# Autodesk Inventor assembly: Rebuild Shooter Assembly
(part 2 of 2)
- Insert:168: Bearing Mount v1:1 ↔ 91831A411:4
- Insert:169: Bearing Mount v1:1 ↔ 91831A411:5
- Insert:170: Bearing Mount v1:1 ↔ 91831A411:6
- Insert:171: Runner Rails v2:1 ↔ 91735A831:1
- Insert:172: Runner Rails v2:1 ↔ 91735A831:2
- Insert:173: Runner Rails v2:1 ↔ 91735A831:3
- Insert:174: Runner Rails v2:1 ↔ 91735A831:4
- Insert:175: Runner Rails v2:1 ↔ 91735A831:6
- Insert:176: Runner Rails v2:1 ↔ 91735A831:5
- Mate:119: Shooter Top Shield:1 ↔ Shooter Magnetic Sensor Mount Bracket:1
- Angle:74 (5 deg): Shooter Magnetic Sensor Mount Bracket:1 ↔ Bearing Mount Top:1
- Mate:120: Shooter Magnetic Sensor Mount Bracket:1 ↔ Bearing Mount Top:1
- Mate:121 (12.7 mm): Shooter Magnetic Sensor Mount Bracket:1 ↔ Bearing Mount Top:1
- Insert:177: Shooter Magnetic Sensor Mount Bracket:1 ↔ Shooter Magnetic Sensor V2:1
- Insert:178: Shooter Magnetic Sensor Mount Bracket:1 ↔ 7:1
- Insert:179: 7:1 ↔ 7:2
- [Insert]: Shooter Magnetic Sensor Mount Bracket:1 ↔ Standard #4 Washer:15
- [Insert]: Shooter Magnetic Sensor Mount Bracket:1 ↔ Standard #4 Washer:16
- Insert:182: Standard #10 Washer:6 ↔ 91831A411:7
- Insert:183: Standard #10 Washer:7 ↔ 91831A411:8
- Insert:184: Standard #10 Washer:8 ↔ 91831A411:9
- Insert:185: Standard #10 Washer:9 ↔ 91831A411:10
- Insert:186: Standard #10 Washer:10 ↔ 91831A411:11
- Insert:187: Standard #10 Washer:11 ↔ 91831A411:12
- Insert:188: Pneumatic Hub:2 ↔ Standard #10 Washer:6
- Insert:189: Pneumatic Hub:2 ↔ Standard #10 Washer:7
- Insert:190: Pneumatic Hub:2 ↔ Standard #10 Washer:8
- Insert:191: Pneumatic Hub:2 ↔ Standard #10 Washer:9
- Insert:192: Pneumatic Hub:2 ↔ Standard #10 Washer:10
- Insert:193: Pneumatic Hub:2 ↔ Standard #10 Washer:11
- Mate:122 (12.7 mm): Bearing Mount Top:1 ↔ Pneumatic Hub:2
- Flush:73: Shooter Top Shield:1 ↔ Bearing Mount Top:1
- Mate:123: Shooter Top Shield:1 ↔ Bearing Mount Top:1
- Flush:74: Shooter Top Shield:1 ↔ Bearing Mount Top:1
- Flush:75: Shooter Top Shield:1 ↔ Bearing Mount Top:1
- Mate:124: Shooter Wheel Shields Connector Bar:1 ↔ Wheel Shield 2:1
- Mate:125: Shooter Wheel Shields Connector Bar:1 ↔ Wheel Shield 1:1
- Flush:76: Shooter Wheel Shields Connector Bar:1 ↔ Wheel Shield 2:1
- Mate:126: Rebuild Shooter Main Base:1 ↔ 0.25x20 Washer:95
- Mate:127: Rebuild L-Channel Strength:1 ↔ 0.25x20 Washer:95
- Insert:194: 0.25x20 Washer:95 ↔ 90630A110:34
- Insert:195: 92620A540:10 ↔ 0.25x20 Washer:63
- Insert:196: DBK_0820Spacer_am-2243 (modified 3):1 ↔ Rebuild Shooter Main Base:1
- [Insert]: Wheel Shield 2:1 ↔ Standard #4 Washer:19
- [Insert]: Wheel Shield 1:1 ↔ Standard #4 Washer:18
- Mate:128: Shooter Wheel Shields Connector Bar:1 ↔ Shooter Side Support Bar - L:1
- Insert:199: Wheel Shield 1:1 ↔ 0.125 Pop Rivet:1
- Insert:200: Wheel Shield 1:1 ↔ 0.125 Pop Rivet:2
- Insert:201: Wheel Shield 2:1 ↔ 0.125 Pop Rivet:3
- Insert:202: Wheel Shield 2:1 ↔ 0.125 Pop Rivet:4
- [Insert]: Wheel Shield 1:1 ↔ Standard #4 Washer:17
- Insert:204: 0.125 Pop Rivet:5 ↔ Hopper Bracing P1:1
- [Insert]: Standard #4 Washer:40 ↔ Hopper Bracing P1:1
- [Insert]: Standard #4 Washer:41 ↔ Hopper Bracing P1:1
- Insert:207: Rebuild Shooter Main Base:1 ↔ 0.25x20 Washer:96
- Insert:208: Rebuild L-Channel Strength:1 ↔ 90630A110:35
- Insert:209: 0.25x20 Washer:96 ↔ 92620A540:11
- Mate:130: Runner Rails v2:1 ↔ Hopper Bracing P2:1
- Mate:132: Runner Rails v2:1 ↔ Hopper Bracing P3:1
- Flush:78 (-6.35 mm): Runner Rails v2:1 ↔ Hopper Bracing P3:1
- Mate:133: Runner Rails v2:1 ↔ Hopper Bracing P2:1
- Flush:79: Hopper Left Side Leg:1 ↔ Hopper Bracing P2:1
- Mate:134: Hopper Left Side Leg:1 ↔ Hopper Bracing P2:1
- Mate:135: Runner Rails v2:1 ↔ Hopper Left Side Leg:1
- Mate:137: Hopper Left Side Leg:1 ↔ Hopper Bracing P3:1
- Mate:138: Hopper Bracing Right Leg P13:1 ↔ Hopper Right Side Leg:1
- Mate:153: Bearing Mount Top:1 ↔ Hopper Right Side Leg:1
- Mate:140: Hopper Left Side:1 ↔ Hopper Left Side Leg:1
- Flush:81: Hopper Bottom:1 ↔ Hopper Left Side:1
- Mate:141: Hopper Bottom:1 ↔ Hopper Back Wedge Side:1
- Mate:142: Hopper Left Side:1 ↔ Hopper Back Wedge Side:1
- Flush:82: Hopper Bottom:1 ↔ Hopper Back Wedge Side:1
- Mate:143: Hopper Bottom:1 ↔ Hopper Left Side:1
- Mate:144: Hopper Bracing Top Left P4:1 ↔ Hopper Top:1
- Flush:83: Hopper Left Side:1 ↔ Hopper Top:1
- Flush:84: Hopper Left Side:1 ↔ Hopper Top:1
- Mate:145: Hopper Bracing Top Left P4:1 ↔ Hopper Left Side:1
- Mate:146: Hopper Bracing Top Left P4:1 ↔ Hopper Left Side:1
- Insert:210: 0.125 Pop Rivet:6 ↔ Hopper Left Side:1
- Insert:211: 0.125 Pop Rivet:7 ↔ Hopper Left Side:1
- Insert:212: 0.125 Pop Rivet:8 ↔ Hopper Left Side:1
- Insert:213: 0.125 Pop Rivet:9 ↔ Hopper Left Side:1
- Insert:214: 0.125 Pop Rivet:10 ↔ Hopper Left Side:1
- Mate:147: Hopper Front:1 ↔ Hopper Bottom:1
- Mate:156: Hopper Front:1 ↔ Hopper Left Side:1
- Mate:148: Hopper Front:1 ↔ Hopper Bracing Front Top P8:1
- Mate:167 (0.7937 mm): Hopper Right:1 ↔ Hopper Top:1
- Mate:150: Hopper Front:1 ↔ Hopper Right:1
- Flush:87: Hopper Front:1 ↔ Hopper Right:1
- Mate:151 (0.7937 mm): Hopper Right:1 ↔ Hopper Right Side Leg:1
- Insert:215: 0.125 Pop Rivet:11 ↔ Hopper Top:1
- Insert:216: 0.125 Pop Rivet:12 ↔ Hopper Top:1
- Mate:152 (114.3 mm): Runner Rails v2:1 ↔ Hopper Left Side:1
- Flush:151: Shooter Back Support Bar:1 ↔ Hopper Back Wedge Side:1
- Insert:217: 0.125 Pop Rivet:13 ↔ Hopper Left Side:1
- Insert:218: 0.125 Pop Rivet:14 ↔ Hopper Left Side:1
- Insert:219: 0.125 Pop Rivet:15 ↔ Hopper Left Side:1
- Insert:220: 0.125 Pop Rivet:16 ↔ Hopper Left Side:1
- Insert:221: 0.125 Pop Rivet:17 ↔ Hopper Left Side:1
- Insert:222: 0.125 Pop Rivet:18 ↔ Hopper Left Side:1
- Mate:154: Hopper Bracing Front Left P5:1 ↔ Hopper Left Side:1
- Mate:155: Hopper Front:1 ↔ Hopper Bracing Front Left P5:1
- Flush:152: Hopper Bracing Front Left P5:1 ↔ Hopper Left Side:1
- Mate:157: Hopper Bracing Top Left P4:1 ↔ Hopper Left Side:1
- Mate:158: Hopper Front:1 ↔ Hopper Bracing Front Bottom P6:1
- Mate:159: Hopper Bracing Front Bottom P6:1 ↔ Hopper Bottom:1
- Flush:153 (25.4 mm): Hopper Bracing Front Bottom P6:1 ↔ Hopper Bottom:1
- Insert:223: 0.125 Pop Rivet:19 ↔ Hopper Bottom:1
- Insert:224: 0.125 Pop Rivet:20 ↔ Hopper Bottom:1
- Insert:225: 0.125 Pop Rivet:21 ↔ Hopper Bottom:1
- Insert:226: 0.125 Pop Rivet:22 ↔ Hopper Bottom:1
- Mate:160: Hopper Front:1 ↔ Hopper Bracing Front Right P7:1
- Mate:161: Hopper Right:1 ↔ Hopper Bracing Front Right P7:1
- Mate:162: Hopper Bracing Front Right P7:1 ↔ Hopper Top:1
- Mate:163: Hopper Bracing Front Top P8:1 ↔ Hopper Top:1
- Mate:164: Hopper Front:1 ↔ Hopper Bracing Front Top P8:1
- Flush:154 (25.4 mm): Hopper Right:1 ↔ Hopper Bracing Front Top P8:1
- Mate:165: Hopper Right:1 ↔ Hopper Bracing Right Bottom P9:1
- Mate:166: Hopper Bracing Right Bottom P9:1 ↔ Hopper Bottom:1
- Flush:155: Hopper Bracing Right Bottom P9:1 ↔ Hopper Right Side Leg:1
- Mate:168: Hopper Right:1 ↔ Hopper Bracing Right Top P10:1
- Mate:169: Hopper Bracing Right Top P10:1 ↔ Hopper Top:1
- Flush:156: Hopper Bracing Right Top P10:1 ↔ Hopper Right Side Leg:1
- Mate:170: Hopper Teflon Strip P1:1 ↔ Hopper Bottom:1
- Flush:157 (31.75 mm): Hopper Teflon Strip P1:1 ↔ Hopper Bottom:1
- Mate:171: Hopper Teflon Strip P1:1 ↔ Hopper Bottom:1
- Mate:172: Hopper Teflon Strip P2:1 ↔ Hopper Bottom:1
- Flush:158 (98.425 mm): Hopper Teflon Strip P2:1 ↔ Hopper Bottom:1
- Mate:173: Hopper Teflon Strip P2:1 ↔ Hopper Bottom:1
- Mate:174: Hopper Teflon Strip P3:1 ↔ Hopper Bottom:1
- Flush:159 (171.45 mm): Hopper Teflon Strip P3:1 ↔ Hopper Bottom:1
- Mate:175: Hopper Teflon Strip P3:1 ↔ Hopper Bottom:1
- Mate:176: Hopper Teflon Strip P4:1 ↔ Hopper Bottom:1
- Flush:160 (241.3 mm): Hopper Teflon Strip P4:1 ↔ Hopper Bottom:1
- Mate:177: Hopper Teflon Strip P4:1 ↔ Hopper Bottom:1
- Insert:227: 0.125 Pop Rivet:23 ↔ Hopper Right:1
- Insert:228: 0.125 Pop Rivet:24 ↔ Hopper Right:1
- Insert:229: 0.125 Pop Rivet:25 ↔ Hopper Right:1
- Insert:230: 0.125 Pop Rivet:26 ↔ Hopper Right:1
- Insert:231: 0.125 Pop Rivet:27 ↔ Hopper Right:1
- Insert:232: 0.125 Pop Rivet:28 ↔ Hopper Right:1
- Insert:233: 0.125 Pop Rivet:29 ↔ Hopper Right:1
- Insert:234: 0.125 Pop Rivet:30 ↔ Hopper Right:1
- Insert:235: 0.125 Pop Rivet:31 ↔ Hopper Right:1
- Insert:236: 0.125 Pop Rivet:32 ↔ Hopper Right:1
- Insert:237: 0.125 Pop Rivet:33 ↔ Hopper Right:1
- Insert:238: 0.125 Pop Rivet:34 ↔ Hopper Right:1
- Insert:239: 0.125 Pop Rivet:35 ↔ Hopper Right:1
- Insert:240: 0.125 Pop Rivet:36 ↔ Hopper Right:1
- Insert:241: 0.125 Pop Rivet:37 ↔ Hopper Right:1
- Insert:242: 0.125 Pop Rivet:38 ↔ Hopper Right:1
- Insert:243: 0.125 Pop Rivet:39 ↔ Hopper Top:1
- Insert:244: 0.125 Pop Rivet:40 ↔ Hopper Top:1
- Insert:245: 0.125 Pop Rivet:41 ↔ Hopper Top:1
- Insert:246: 0.125 Pop Rivet:42 ↔ Hopper Top:1
- Insert:247: 0.125 Pop Rivet:43 ↔ Hopper Top:1
- Insert:248: 0.125 Pop Rivet:44 ↔ Hopper Top:1
- Insert:249: 0.125 Pop Rivet:45 ↔ Hopper Top:1
- Flush:161: Hopper Bracing Right Bottom P9:1 ↔ Hopper Bottom:1
- Mate:178: 0.125 Pop Rivet:46 ↔ Hopper Bottom:1
- Mate:179: 0.125 Pop Rivet:47 ↔ Hopper Bottom:1
- Mate:180: 0.125 Pop Rivet:48 ↔ Hopper Bottom:1
- Mate:181: 0.125 Pop Rivet:49 ↔ Hopper Bottom:1
- Mate:182: 0.125 Pop Rivet:50 ↔ Hopper Bottom:1
- Tangent:89: 0.125 Pop Rivet:50 ↔ Hopper Bottom:1
- Tangent:90: 0.125 Pop Rivet:49 ↔ Hopper Bottom:1
- Tangent:91: 0.125 Pop Rivet:48 ↔ Hopper Bottom:1
- Tangent:92: 0.125 Pop Rivet:47 ↔ Hopper Bottom:1
- Tangent:93: 0.125 Pop Rivet:46 ↔ Hopper Bottom:1
- Insert:250: 0.125 Pop Rivet:51 ↔ Hopper Right:1
- Insert:251: 0.125 Pop Rivet:52 ↔ Hopper Right:1
- Insert:252: 0.125 Pop Rivet:53 ↔ Hopper Front:1
- Insert:253: 0.125 Pop Rivet:54 ↔ Hopper Front:1
- Insert:254: 0.125 Pop Rivet:55 ↔ Hopper Front:1
- Insert:255: 0.125 Pop Rivet:56 ↔ Hopper Front:1
- Insert:256: 0.125 Pop Rivet:57 ↔ Hopper Front:1
- Insert:257: 0.125 Pop Rivet:58 ↔ Hopper Front:1
- Insert:258: 0.125 Pop Rivet:59 ↔ Hopper Front:1
- Insert:259: 0.125 Pop Rivet:60 ↔ Hopper Front:1
- Insert:260: 0.125 Pop Rivet:61 ↔ Hopper Front:1
- Insert:261: 0.125 Pop Rivet:62 ↔ Hopper Front:1
- Insert:262: 0.125 Pop Rivet:63 ↔ Hopper Front:1
- Insert:263: 0.125 Pop Rivet:64 ↔ Hopper Front:1
- Insert:264: 0.125 Pop Rivet:65 ↔ Hopper Left Side:1
- Insert:265: 0.125 Pop Rivet:66 ↔ Hopper Left Side:1
- Insert:266: 0.125 Pop Rivet:67 ↔ Hopper Left Side:1
- Mate:183: Hopper Bracing Back Bottom P11:1 ↔ Hopper Bottom:1
- Mate:184: Hopper Bracing Back Bottom P11:1 ↔ Hopper Back Wedge Side:1
- Mate:185: Hopper Bracing Back Left P12:1 ↔ Hopper Left Side:1
- Mate:186: Hopper Bracing Back Left P12:1 ↔ Hopper Back Wedge Side:1
- Flush:162 (-6.35 mm): Hopper Bracing Back Left P12:1 ↔ Hopper Back Wedge Side:1
- Mate:187 (6.35 mm): Hopper Bracing Back Bottom P11:1 ↔ Hopper Bracing Back Left P12:1
- Insert:267: 0.125 Pop Rivet:68 ↔ Hopper Back Wedge Side:1
- Insert:268: 0.125 Pop Rivet:69 ↔ Hopper Back Wedge Side:1
- Insert:269: 0.125 Pop Rivet:70 ↔ Hopper Back Wedge Side:1
- Insert:270: 0.125 Pop Rivet:71 ↔ Hopper Back Wedge Side:1
- Insert:271: 0.125 Pop Rivet:72 ↔ Hopper Back Wedge Side:1
- Insert:272: 0.125 Pop Rivet:73 ↔ Hopper Back Wedge Side:1
- Insert:273: 0.125 Pop Rivet:74 ↔ Hopper Back Wedge Side:1
- Insert:274: 0.125 Pop Rivet:75 ↔ Hopper Back Wedge Side:1
- Mate:188: Shooter Top Shield:1 ↔ Hopper Bracing Right Leg P13:1
- Mate:189: Hopper Bracing Right Leg P13:1 ↔ Hopper Right Side Leg:1
- Flush:163: Shooter Top Shield:1 ↔ Hopper Bracing Right Leg P13:1
- Insert:275: 0.125 Pop Rivet:76 ↔ Hopper Left Side:1
- Insert:276: 0.125 Pop Rivet:77 ↔ Hopper Left Side:1
- Insert:277: Standard #4 Washer:6 ↔ Hopper Right Side Leg:1
- Insert:278: Standard #4 Washer:7 ↔ Hopper Right Side Leg:1
- Insert:279: Standard #4 Washer:8 ↔ Hopper Right Side Leg:1
- [Insert]: Standard #4 Washer:10 ↔ Hopper Bracing Right Leg P13:1
- [Insert]: Standard #4 Washer:9 ↔ Hopper Bracing Right Leg P13:1
- [Insert]: Standard #4 Washer:32 ↔ Hopper Bracing P2:1
- Insert:284: Standard #4 Washer:31 ↔ Hopper Left Side Leg:1
- [Insert]: Standard #4 Washer:30 ↔ Hopper Bracing P2:1
- Insert:286: Standard #4 Washer:29 ↔ Hopper Left Side Leg:1
- [Insert]: Standard #4 Washer:25 ↔ Hopper Bracing P3:1
- [Insert]: Standard #4 Washer:26 ↔ Hopper Bracing P3:1
- [Insert]: Standard #4 Washer:27 ↔ Hopper Bracing P3:1
- Insert:290: Standard #4 Washer:24 ↔ Hopper Left Side Leg:1
- Insert:291: Standard #4 Washer:28 ↔ Hopper Left Side Leg:1
- Mate:190: Hopper Bouncer Mounting Brace P1:2 ↔ Hopper Front:1
- Mate:191: Hopper Bouncer Mounting Brace P1:1 ↔ Hopper Front:1
- Mate:194 (152.4 mm): Hopper Bouncer Mounting Brace P1:1 ↔ Hopper Bouncer Mounting Brace P1:2
- Mate:195 (215.9 mm): Hopper Bouncer Mounting Brace P1:2 ↔ Hopper Right:1
- Mate:196 (107.95 mm): Hopper Bouncer Mounting Brace P1:2 ↔ Hopper Top:1
- Flush:164: Hopper Bouncer Mounting Brace P1:1 ↔ Hopper Bouncer Mounting Brace P1:2
- Insert:292: 0.125 Pop Rivet:78 ↔ Bounce Polycarbonate Flap:1
- Insert:293: 0.125 Pop Rivet:79 ↔ Bounce Polycarbonate Flap:1
- Insert:294: 0.125 Pop Rivet:80 ↔ Bounce Polycarbonate Flap:1
- Insert:295: 0.125 Pop Rivet:81 ↔ Hopper Bouncer Mounting Brace P1:2
- Insert:296: 0.125 Pop Rivet:82 ↔ Hopper Bouncer Mounting Brace P1:1
- Insert:297: 0.125 Pop Rivet:84 ↔ Hopper Bouncer Mounting Brace P1:1
- Insert:298: 0.125 Pop Rivet:83 ↔ Hopper Bouncer Mounting Brace P1:2
- Mate:197: 0.125 Pop Rivet:78 ↔ Hopper Top:1
- Mate:198: 0.125 Pop Rivet:80 ↔ Hopper Top:1
- Mate:199: Bounce Polycarbonate Flap:1 ↔ Hopper Top:1
- Mate:200: Runner Rails v2:1 ↔ Trimmed Leaktite 3.5-Gal. Blue Plastic Translucent Pail Hopper V3:1
- Tangent:94 (31.75 mm): Runner Rails v2:1 ↔ Trimmed Leaktite 3.5-Gal. Blue Plastic Translucent Pail Hopper V3:1
- Flush:165 (190.5 mm): Runner Rails v2:1 ↔ Trimmed Leaktite 3.5-Gal. Blue Plastic Translucent Pail Hopper V3:1
- Tangent:202: Hopper Bracing P12 to P1:1 ↔ Trimmed Leaktite 3.5-Gal. Blue Plastic Translucent Pail Hopper V3:1
- Mate:201: Hopper Bracing P12 to P1:1 ↔ Hopper Bracing P1:1
- Mate:202: Runner Rails v2:1 ↔ Hopper Pail Mounting Brace P13:1
- Tangent:203: Hopper Pail Mounting Brace P13:1 ↔ Trimmed Leaktite 3.5-Gal. Blue Plastic Translucent Pail Hopper V3:1
- Mate:203 (2.54 mm): Hopper Pail Mounting Brace P13:1 ↔ Hopper Bracing P3:1
- Mate:204: Hopper Pail Mounting Brace P13:1 ↔ Trimmed Leaktite 3.5-Gal. Blue Plastic Translucent Pail Hopper V3:1
- Insert:299: 0.125 Pop Rivet:85 ↔ Hopper Pail Mounting Brace P13:1
- Mate:205: Runner Rails v2:1 ↔ 0.125 Pop Rivet:85
- Mate:206: Runner Rails v2:1 ↔ Hopper Pail Mounting Brace P13:2
- Tangent:204: Hopper Pail Mounting Brace P13:2 ↔ Trimmed Leaktite 3.5-Gal. Blue Plastic Translucent Pail Hopper V3:1
- Mate:207: Hopper Pail Mounting Brace P13:2 ↔ Trimmed Leaktite 3.5-Gal. Blue Plastic Translucent Pail Hopper V3:1
- Angle:75 (90 deg): Hopper Pail Mounting Brace P13:1 ↔ Hopper Pail Mounting Brace P13:2
- Insert:300: 0.125 Pop Rivet:86 ↔ Hopper Pail Mounting Brace P13:2
- Mate:208: Hopper Teflon Strip P5:1 ↔ Hopper Bottom:1
- Mate:209: Hopper Teflon Strip P5:1 ↔ Hopper Teflon Strip P4:1
- Mate:210: Hopper Teflon Strip P6:1 ↔ Hopper Bottom:1
- Mate:211: Hopper Teflon Strip P6:1 ↔ Hopper Teflon Strip P3:1
- Flush:166 (6.35 mm): Hopper Teflon Strip P5:1 ↔ Hopper Teflon Strip P6:1
- Mate:212 (38.1 mm): Hopper Teflon Strip P6:1 ↔ Hopper Teflon Strip P3:1
- Mate:213: Hopper to Pail Polycarbonate Flap Connector V2:1 ↔ Hopper Front:1
- Insert:301: 0.125 Pop Rivet:88 ↔ Hopper to Pail Polycarbonate Flap Connector V2:1
- Insert:302: 0.125 Pop Rivet:87 ↔ Hopper to Pail Polycarbonate Flap Connector V2:1
- Angle:76 (90 deg): Hopper to Pail Polycarbonate Flap Connector V2:1 ↔ Hopper Top:1
- Mate:214: Hopper to Pail Polycarbonate Flap Connector V2:1 ↔ Trimmed Leaktite 3.5-Gal. Blue Plastic Translucent Pail Hopper V3:1
- Angle:77 (0 deg): Hopper to Pail Polycarbonate Flap Connector V2:1 ↔ Hopper Right:1
- Mate:215 (146.05 mm): Hopper to Pail Polycarbonate Flap Connector V2:1 ↔ Hopper Top:1
- Tangent:207: 0.125 Pop Rivet:5 ↔ Hopper Bracing P12 to P1:1
- Flush:167: Hopper Pail Mounting Brace P13:2 ↔ Trimmed Leaktite 3.5-Gal. Blue Plastic Translucent Pail Hopper V3:1
- Mate:216: 0.125 Pop Rivet:89 ↔ Trimmed Leaktite 3.5-Gal. Blue Plastic Translucent Pail Hopper V3:1
- Tangent:208: 0.125 Pop Rivet:89 ↔ Trimmed Leaktite 3.5-Gal. Blue Plastic Translucent Pail Hopper V3:1
- Flush:168: Hopper Pail Mounting Brace P13:1 ↔ Trimmed Leaktite 3.5-Gal. Blue Plastic Translucent Pail Hopper V3:1
- Mate:217: 0.125 Pop Rivet:90 ↔ Trimmed Leaktite 3.5-Gal. Blue Plastic Translucent Pail Hopper V3:1
- Tangent:209: 0.125 Pop Rivet:90 ↔ Trimmed Leaktite 3.5-Gal. Blue Plastic Translucent Pail Hopper V3:1
- Angle:78 (-85.75 deg): Hopper to Pail Polycarbonate Flap Connector V2:1 ↔ Hopper Top:1
- Mate:218: 0.125 Pop Rivet:87 ↔ Trimmed Leaktite 3.5-Gal. Blue Plastic Translucent Pail Hopper V3:1
- Mate:219: 0.125 Pop Rivet:88 ↔ Hopper Front:1
- Insert:303: Rebuild L-Channel Strength:1 ↔ 91831A005:13
- Insert:304: Rebuild L-Channel Strength:1 ↔ 91831A005:14
- Insert:305: Shooter Side Support Bar - L:1 ↔ 90715A007:3
- [Insert]: 91772A110:8 ↔ Standard #4 Washer:18
- [Insert]: 91772A110:9 ↔ Standard #4 Washer:17
- [Insert]: 91772A110:10 ↔ Standard #4 Washer:19
- Insert:309: 91831A005:15 ↔ Standard #4 Washer:33
- Insert:310: 91831A005:16 ↔ Standard #4 Washer:34
- [Insert]: Runner Rails v2:1 ↔ Standard #4 Washer:33
- [Insert]: Runner Rails v2:1 ↔ Standard #4 Washer:34
- Insert:313: 91831A005:17 ↔ Standard #4 Washer:35
- Insert:314: 91831A005:18 ↔ Standard #4 Washer:36
- Insert:315: 91831A005:19 ↔ Standard #4 Washer:37
- [Insert]: Runner Rails v2:1 ↔ Standard #4 Washer:35
- [Insert]: Runner Rails v2:1 ↔ Standard #4 Washer:36
- [Insert]: Runner Rails v2:1 ↔ Standard #4 Washer:37
- [Insert]: 91772A112:4 ↔ Standard #4 Washer:25
- [Insert]: 91772A112:5 ↔ Standard #4 Washer:26
- [Insert]: 91772A112:6 ↔ Standard #4 Washer:27
- [Insert]: 91772A112:7 ↔ Standard #4 Washer:30
- [Insert]: 91772A112:8 ↔ Standard #4 Washer:32
- Insert:324: 91831A005:9 ↔ Standard #4 Washer:20
- Insert:325: 91831A005:10 ↔ Standard #4 Washer:21
- Insert:326: 91831A005:11 ↔ Standard #4 Washer:22
- Insert:327: 91831A005:12 ↔ Standard #4 Washer:23
- Insert:328: Standard #4 Washer:20 ↔ Hopper Bracing P2:1
- Insert:329: Standard #4 Washer:21 ↔ Hopper Bracing P2:1
- Insert:330: Standard #4 Washer:22 ↔ Hopper Bracing P3:1
- Insert:331: Standard #4 Washer:23 ↔ Hopper Bracing P3:1
- [Insert]: 91772A110:7 ↔ Standard #4 Washer:31
- [Insert]: 91772A110:6 ↔ Standard #4 Washer:29
- [Insert]: 91772A110:5 ↔ Standard #4 Washer:28
- [Insert]: 91772A110:4 ↔ Standard #4 Washer:24
- Insert:336: 91257A544:3 ↔ 0.25x20 Washer:62
- Insert:337: 91831A005:4 ↔ Standard #4 Washer:5
- Insert:338: 91831A005:5 ↔ Standard #4 Washer:4
- Insert:339: 91831A005:6 ↔ Standard #4 Washer:3
- Insert:340: Standard #4 Washer:5 ↔ Hopper Bracing Right Leg P13:1
- Insert:341: Standard #4 Washer:4 ↔ Hopper Bracing Right Leg P13:1
- Insert:342: Standard #4 Washer:3 ↔ Hopper Bracing Right Leg P13:1
- [Insert]: 91772A110:1 ↔ Standard #4 Washer:6
- [Insert]: 91772A110:2 ↔ Standard #4 Washer:7
- [Insert]: 91772A110:3 ↔ Standard #4 Washer:8
- Insert:346: 91831A005:2 ↔ Standard #4 Washer:11
- [Insert]: Bearing Mount Top:1 ↔ Standard #4 Washer:11
- Insert:348: 91831A005:3 ↔ Standard #4 Washer:12
- [Insert]: Bearing Mount Top:1 ↔ Standard #4 Washer:12
- [Insert]: 91772A112:2 ↔ Standard #4 Washer:10
- [Insert]: 91772A112:3 ↔ Standard #4 Washer:9
- [Insert]: 91831A005:21 ↔ Standard #4 Washer:39
- [Insert]: 91831A005:20 ↔ Standard #4 Washer:38
- [Insert]: Runner Rails v2:1 ↔ Standard #4 Washer:39
- [Insert]: Runner Rails v2:1 ↔ Standard #4 Washer:38
- [Insert]: 91772A112:9 ↔ Standard #4 Washer:40
- [Insert]: 91772A112:10 ↔ Standard #4 Washer:41
- Mate:221 (-16.51 mm): Runner Rails v2:1 ↔ Hopper Bracing P1:1
- Mate:222 (2.54 mm): Rebuild Outer Rail v1:5 ↔ Hopper Bracing P1:1
- Mate:223 (25.4 mm): Hopper Bracing P12 to P1:1 ↔ Hopper Bracing P1:1
- Flush:170 (3.175 mm): Hopper Bracing P12 to P1:1 ↔ Hopper Bracing P1:1
- Flush:171: Hopper Bracing P12 to P1:1 ↔ Hopper Bracing P1:1
- Flush:172: Hopper Bracing P12 to P1:1 ↔ Trimmed Leaktite 3.5-Gal. Blue Plastic Translucent Pail Hopper V3:1
- Mate:224: 0.125 Pop Rivet:91 ↔ Trimmed Leaktite 3.5-Gal. Blue Plastic Translucent Pail Hopper V3:1
- Tangent:211: 0.125 Pop Rivet:91 ↔ Trimmed Leaktite 3.5-Gal. Blue Plastic Translucent Pail Hopper V3:1
- Insert:358: DBK_0820Spacer_am-2243 (modified for Shooter Shaft Spacer 1):1 ↔ CIM Bearing:2
- Insert:359: DBK_0820Spacer_am-2243 (modified for Shooter Shaft Spacer 2):1 ↔ Pneumatic Hub:2
- [Insert]: 91257A544:4 ↔ 0.25x20 Washer:97
- Insert:361: Shooter Side Support Bar - L:1 ↔ 0.25x20 Washer:97
- Insert:362: DBK_0820Spacer_am-2243 (modified 2):2 ↔ 0.25x20 Washer:27
- Insert:363: Cim Mount:1 ↔ Standard #10 Washer:13
- Insert:364: Cim Mount:1 ↔ Standard #10 Washer:12
- Insert:365: Standard #10 Washer:12 ↔ 91251A345:2
- Insert:366: Standard #10 Washer:13 ↔ 91251A345:1
- Insert:367: 91251A355:1 ↔ Standard #10 Washer:14
- Insert:368: Pneumatic Hub:1 ↔ Standard #10 Washer:14
- [Insert]: 91251A355:2 ↔ Standard #10 Washer:15
- [Insert]: 91251A355:3 ↔ Standard #10 Washer:16
- [Insert]: 91251A355:4 ↔ Standard #10 Washer:17
- [Insert]: 91251A355:5 ↔ Standard #10 Washer:18
- [Insert]: 91251A355:6 ↔ Standard #10 Washer:19
- Insert:374: Pneumatic Hub:1 ↔ Standard #10 Washer:15
- Insert:375: Pneumatic Hub:1 ↔ Standard #10 Washer:16
- Insert:376: Pneumatic Hub:1 ↔ Standard #10 Washer:17
- Insert:377: Pneumatic Hub:1 ↔ Standard #10 Washer:19
- Insert:378: Pneumatic Hub:1 ↔ Standard #10 Washer:18
- Insert:379: 91831A005:8 ↔ Standard #4 Washer:14
- Insert:380: 91831A005:7 ↔ Standard #4 Washer:13
- [Insert]: Bearing Mount Top:1 ↔ Standard #4 Washer:14
- [Insert]: Bearing Mount Top:1 ↔ Standard #4 Washer:13
- [Insert]: 91772A113:1 ↔ Standard #4 Washer:15
- [Insert]: 91772A113:2 ↔ Standard #4 Washer:16
- Flush:173: Shooter 8mm Key Primary Wheel:1 ↔ Pneumatic Hub:2
- Mate:225: Shooter 8mm Key Primary Wheel:1 ↔ Pneumatic Hub:2
- Mate:226: Shooter 8mm Key Primary Wheel:1 ↔ 8mm shaft 2:1
- Mate:227: Shooter 8mm Key Primary Wheel:1 ↔ Pneumatic Hub:2
- Mate:228: Shooter Side Support Bar - L:1 ↔ Rebuild Shooter NCDME075-0600 Cylinder Mounting Bracket:1
- Mate:229 (2.032 mm): Shooter Side Support Bar - L:1 ↔ Rebuild Shooter NCDME075-0600 Cylinder Mounting Bracket:1
- Insert:385: NCDME075-0600 SMC Pneumatic Cylinder:1 ↔ Rebuild Shooter NCDME075-0600 Cylinder Mounting Bracket:1
- Angle:79 (270 deg): Rebuild Shooter Main Base:1 ↔ NCDME075-0600 SMC Pneumatic Cylinder:1
- Flush:174 (170.18 mm): Shooter Back Support Bar:1 ↔ Rebuild Shooter NCDME075-0600 Cylinder Mounting Bracket:1
- Insert:386: 94846A535:1 ↔ Rebuild Shooter NCDME075-0600 Cylinder Mounting Bracket:1
- Flush:175 (-21.336 mm): Shooter I Brace:1 ↔ NCDME075-0600 SMC Pneumatic Cylinder:1
- [Insert]: 90630A110:36 ↔ 0.25x20 Washer:98
- Insert:388: 0.25x20 Washer:98 ↔ NCDME075-0600 SMC Pneumatic Cylinder:1
- Insert:389: 91257A544:5 ↔ 0.25x20 Washer:99
- Insert:390: Shooter I Brace:1 ↔ 0.25x20 Washer:99
- Flush:176 (-186.182 mm): Shooter Side Support Bar - L:1 ↔ NCDME075-0600 SMC Pneumatic Cylinder:1
- Mate:230: Rebuild Puller Hook:1 ↔ NCDME075-0600 SMC Pneumatic Cylinder:1
- Flush:177 (7.62 mm): Rebuild Puller Hook:1 ↔ NCDME075-0600 SMC Pneumatic Cylinder:1
- Angle:80 (0 deg): Rebuild Shooter Main Base:1 ↔ Rebuild Puller Hook:1
- Insert:391: 90630A110:37 ↔ Rebuild Puller Hook:1
- Insert:392: Shooter I Brace:1 ↔ 0.25x20 Washer:100
- Insert:393: Shooter I Brace:1 ↔ 0.25x20 Washer:101
- Insert:394: Shooter I Brace:1 ↔ 0.25x20 Washer:102
- Insert:395: Spur Gear2:1 ↔ Standard #4 Washer:1
- Insert:396: Spur Gear2:1 ↔ Standard #4 Washer:2
- Insert:397: Standard #4 Washer:2 ↔ 91831A005:1
- Insert:398: Standard #4 Washer:1 ↔ 91772A112:1
## Named parameters: d115_d109 = 0 mm, d120_d109 = 0 mm, d128_d126 = 0 mm, d130_d128_d126 = 0 mm, d282_d280 = 0 mm, d284_d279 = 0 mm, d286_d279 = 0 mm, d288_d163 = 0 mm, d290_d163 = 0 mm, d291_d163 = 0 mm, d292_d163 = 0 mm, d308_d280 = 0 mm, d311_d280 = 0 mm, d314_d280 = 0 mm, d642_d638 = 0 mm, d643_d638 = 0 mm, d644_d638 = 0 mm, d653_d638 = 0 mm, d654_d638 = 0 mm, d655_d638 = 0 mm, d656_d638 = 0 mm, d666_d653_d638 = 0 mm, d667_d653_d638 = 0 mm, d668_d653_d638 = 0 mm, d675_d666_d653_d638 = 0 mm, d677_d666_d653_d638 = 0 mm, d681_d656_d638 = 0 mm, d682_d656_d638 = 0 mm, d697_d665 = 0 mm, d706_d704 = 0 mm, d707_d704 = 0 mm, d708_d704 = 0 mm, d709_d704 = 0 mm, d710_d704 = 0 mm, d716_d653_d638 = 0 mm, d717_d653_d638 = 0 mm, d733_d290_d163 = 0 mm
